# Autodesk Inventor assembly: Conveyer Boat
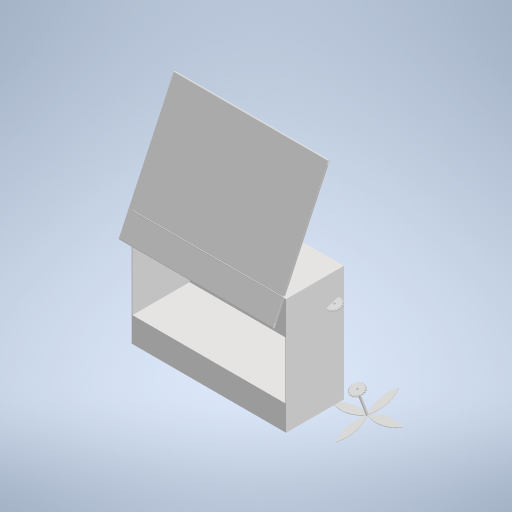
[picture p0: Inventor's stored thumbnail of the model, 512x512]
Saved by Autodesk Inventor 2024 (Build 280153000, 153)
## iProperties
Created: 2024-09-16
Part Number: Conveyer Boat
Document SubType Name: Assembly
Designer: srira
Author: srira
## Documents named in this file (5)
- C:\Users\srira\Documents\IITGN\3rd year\Sem5\ES408\Tentative Model\Conveyer Boat.iam
- C:\Users\srira\Documents\IITGN\3rd year\Sem5\ES408\Tentative Model\Conveyer Belt.ipt
- C:\Users\srira\Documents\IITGN\3rd year\Sem5\ES408\Tentative Model\Top Bin.ipt
- C:\Users\srira\Documents\IITGN\3rd year\Sem5\ES408\Tentative Model\Ger.ipt
- C:\Users\srira\Documents\IITGN\3rd year\Sem5\ES408\Tentative Model\ranpro.ipt
## Components (8 placed, 4 different names)
1. Conveyer Belt:1
2. Top Bin:1
3. Ger:1 — Mate:1, Insert:1
4. Ger:2 — Mate:1
5. Ger:3 — Mate:2
6. Ger:4 — Mate:2, Insert:2
7. ranpro:1 — Insert:1
8. ranpro:2 — Insert:2
## Relationships (4: Mate 2, Insert 2)
- Mate:1: Ger:1 ↔ Ger:2
- Insert:1: Ger:1 ↔ ranpro:1
- Mate:2: Ger:3 ↔ Ger:4
- Insert:2: Ger:4 ↔ ranpro:2
